# Autodesk Inventor assembly: STAGE1,ELEVATOR
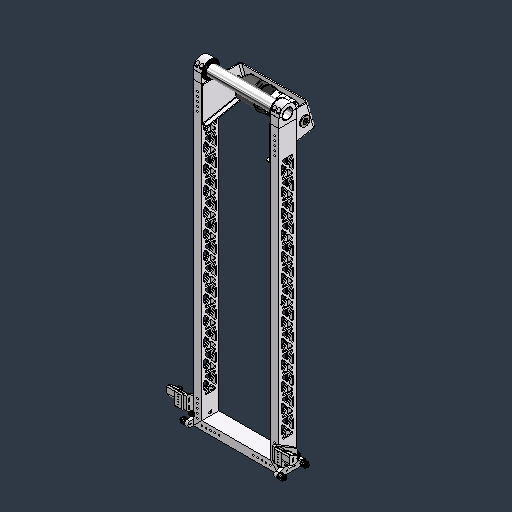
[picture p0: Inventor's stored thumbnail of the model, 512x512]
Saved by Autodesk Inventor 2024.3 (Build 283343000, 343)
## iProperties
ILogicPurgeVersion: 0.0.0.0
OnSaveVersion: 3.5.0.0
OnSaveAssembly: COREAutomationManager
Created: 2025-02-04
Part Number: STAGE1,ELEVATOR
Document SubType Name: Assembly
Designer: Jthib
Mfg Approved By: John.Thibert
Mass: 2890.66 g
Surface Area: 6308.95 cm^2
Volume: 985.653 cm^3
Density: 2.93273 g/cm^3
ModelCat: Uncategorized
CN_MASS: 2.89
Author: Jthib
## Documents named in this file (22)
- D:\Inventor Projects\Poseidon V2\STAGE1,ELEVATOR.iam
- D:\Inventor Projects\Poseidon V2\TUBE,ELEVATOR,SIDE,STAGE1.ipt
- D:\Inventor Projects\Poseidon V2\TUBE,ELEVATOR,BOT,STAGE1.ipt
- D:\Inventor Projects\Poseidon V2\PLATE,BRACKET,ELEVATOR,STAGE1.ipt
- D:\Inventor Projects\Poseidon V2\SLIDE,ELEVATOR,STAGE1,LH.iam
- D:\Inventor Projects\Poseidon V2\SLIDE,ELEVATOR,STAGE1,RH.iam
- D:\Inventor Projects\Poseidon V2\BRACE,CHAIN,#25,ELEVATOR.ipt
- D:\Inventor Projects\Poseidon V2\60355K336_Ball Bearing.ipt
- D:\Inventor Projects\Poseidon V2\91259A171_Alloy Steel Shoulder Screw.ipt
- D:\Inventor Projects\Poseidon V2\BEARING,MOUNT,SIDE,ELEVATOR,MIRR.ipt
- D:\Inventor Projects\Poseidon V2\BEARING,MOUNT,SIDE,ELEVATOR.ipt
- D:\Inventor Projects\Poseidon V2\BLOCK,BEARING,ARM,ELEVATOR.ipt
- D:\Inventor Projects\Poseidon V2\TOP,BEARING_BLOCK,ELEVATOR.ipt
- D:\Inventor Projects\Poseidon V2\TUBE,AXLE,ARM.ipt
- D:\Inventor Projects\Poseidon V2\PLATE,CROSSBRACE,MOTOR,ARM.ipt
- D:\Inventor Projects\Poseidon V2\Purchased\5909K52_0.032 Thick Washer for 1-1-4 Shaft Diameter Needle-Roller Thrust Bearing\5909K52_0.032 Thick Washer for 1-1-4 Shaft Diameter Needle-Rol.ipt
- D:\Inventor Projects\Poseidon V2\Purchased\5909K38_Needle-Roller Thrust Bearing\5909K38_Needle-Roller Thrust Bearing\5909K38_Needle-Roller Thrust Bearing.ipt
- D:\Inventor Projects\Poseidon V2\PURCHASED,HEX_BEARING.ipt
- D:\Inventor Projects\Poseidon V2\#Poseidon 2025\Design Accelerator\Spur Gear13.ipt
- D:\Inventor Projects\Poseidon V2\VersaPlanetary v2 Dual Stage 10_1 with RS 550 (1).iam
- D:\Inventor Projects\Poseidon V2\CONTROLS,MOTOR,NEO,V1.ipt
- D:\Inventor Projects\Poseidon V2\1_CAD Library\PURCHASED,GEARBOX,VERSA_PLANETARY,ADAPTER_CIM.ipt
## Components (35 placed, 23 different names)
1. 5909K38_Needle-Roller Thrust Bearing:1
2. 5909K38_Needle-Roller Thrust Bearing:2
3. 5909K52_0.032 Thick Washer for 1-1-4 Shaft Diameter Needle-Rol:1
4. 5909K52_0.032 Thick Washer for 1-1-4 Shaft Diameter Needle-Rol:2
5. 5909K52_0.032 Thick Washer for 1-1-4 Shaft Diameter Needle-Rol:3
6. 5909K52_0.032 Thick Washer for 1-1-4 Shaft Diameter Needle-Rol:4
7. 60355K336_Ball Bearing:1
8. 60355K336_Ball Bearing:2
9. 91259A171_Alloy Steel Shoulder Screw:1
10. 91259A171_Alloy Steel Shoulder Screw:2
11. BEARING,MOUNT,SIDE,ELEVATOR,MIRR:1
12. BEARING,MOUNT,SIDE,ELEVATOR:1
13. BLOCK,BEARING,ARM,ELEVATOR:1 — Mate:51, Mate:52, Mate:53, Mate:54, Mate:58, Mate:59
14. BLOCK,BEARING,ARM,ELEVATOR:3 — Mate:55, Mate:56, Mate:57, Mate:60, Mate:61
15. BRACE,CHAIN,#25,ELEVATOR.ipt:1
16. BRACE,CHAIN,#25,ELEVATOR:2 — Mate:16, Mate:17, Mate:18
17. CONTROLS,MOTOR,NEO,V1:1
18. PLATE,BRACKET,ELEVATOR,STAGE1.ipt:1
19. PLATE,BRACKET,ELEVATOR,STAGE1.ipt:2 — Mate:42, Mate:44
20. PLATE,BRACKET,ELEVATOR,STAGE1:4 — Mate:19, Mate:20, Mate:48, Mate:49, Mate:50
21. PLATE,BRACKET,ELEVATOR,STAGE1:5 — Mate:22, Mate:23, Mate:41, Mate:43, Mate:45, Mate:47
22. PLATE,CROSSBRACE,MOTOR,ARM:1
23. PURCHASED,GEARBOX,VERSA_PLANETARY,ADAPTER_CIM:1
24. PURCHASED,HEX_BEARING:1 — Mate:80
25. SLIDE,ELEVATOR,STAGE1,LH.iam:1 [sub-assembly] — Mate:15, Mate:16, Mate:17, Mate:18
26. SLIDE,ELEVATOR,STAGE1,RH.iam:1 [sub-assembly] — Mate:46
27. Spur Gear1:1 — Mate:80
28. TOP,BEARING_BLOCK,ELEVATOR:1 — Mate:58, Mate:59
29. TOP,BEARING_BLOCK,ELEVATOR:2 — Mate:60, Mate:61
30. TUBE,AXLE,ARM:1
31. TUBE,ELEVATOR,BOT,STAGE1.ipt:1 — Mate:14, Mate:19, Mate:20, Mate:22, Mate:23, Mate:41, Mate:42
32. TUBE,ELEVATOR,SIDE,STAGE1.ipt:1 — Mate:13, Mate:48, Mate:49, Mate:50, Mate:51, Mate:52, Mate:53, Mate:54
33. TUBE,ELEVATOR,SIDE,STAGE1.ipt:2 — Mate:43, Mate:44, Mate:45, Mate:46, Mate:47, Mate:55, Mate:56, Mate:57
34. TUBE,AXLE,ARM:2
35. VersaPlanetary v2 Dual Stage 10_1 with RS 550 (1):1 [sub-assembly]
## Relationships (82: Mate 67, Insert 8, Tangent 4, Flush 3)
- [Insert]: PLATE,BRACKET,ELEVATOR,STAGE1.ipt:1 ↔ TUBE,ELEVATOR,BOT,STAGE1.ipt:1
- [Insert]: PLATE,BRACKET,ELEVATOR,STAGE1.ipt:1 ↔ TUBE,ELEVATOR,BOT,STAGE1.ipt:1
- [Insert]: PLATE,BRACKET,ELEVATOR,STAGE1.ipt:2 ↔ TUBE,ELEVATOR,BOT,STAGE1.ipt:1
- [Insert]: PLATE,BRACKET,ELEVATOR,STAGE1.ipt:2 ↔ TUBE,ELEVATOR,BOT,STAGE1.ipt:1
- [Mate]: SLIDE,ELEVATOR,STAGE1,RH.iam:1 ↔ TUBE,ELEVATOR,SIDE,STAGE1.ipt:2
- [Mate]: SLIDE,ELEVATOR,STAGE1,RH.iam:1 ↔ TUBE,ELEVATOR,SIDE,STAGE1.ipt:2
- [Mate]: SLIDE,ELEVATOR,STAGE1,LH.iam:1 ↔ TUBE,ELEVATOR,SIDE,STAGE1.ipt:1
- [Mate]: SLIDE,ELEVATOR,STAGE1,LH.iam:1 ↔ TUBE,ELEVATOR,SIDE,STAGE1.ipt:1
- [Mate]: BRACE,CHAIN,#25,ELEVATOR.ipt:1 ↔ SLIDE,ELEVATOR,STAGE1,RH.iam:1
- [Mate]: BRACE,CHAIN,#25,ELEVATOR.ipt:1 ↔ SLIDE,ELEVATOR,STAGE1,RH.iam:1
- [Mate]: BRACE,CHAIN,#25,ELEVATOR.ipt:1 ↔ SLIDE,ELEVATOR,STAGE1,RH.iam:1
- Mate:13 (-127 mm): TUBE,ELEVATOR,SIDE,STAGE1.ipt:1
- Mate:14 (-457.2 mm): TUBE,ELEVATOR,BOT,STAGE1.ipt:1
- Mate:15: SLIDE,ELEVATOR,STAGE1,LH.iam:1
- Mate:16: BRACE,CHAIN,#25,ELEVATOR:2 ↔ SLIDE,ELEVATOR,STAGE1,LH.iam:1
- Mate:17: BRACE,CHAIN,#25,ELEVATOR:2 ↔ SLIDE,ELEVATOR,STAGE1,LH.iam:1
- Mate:18: BRACE,CHAIN,#25,ELEVATOR:2 ↔ SLIDE,ELEVATOR,STAGE1,LH.iam:1
- Mate:19: PLATE,BRACKET,ELEVATOR,STAGE1:4 ↔ TUBE,ELEVATOR,BOT,STAGE1.ipt:1
- Mate:20: PLATE,BRACKET,ELEVATOR,STAGE1:4 ↔ TUBE,ELEVATOR,BOT,STAGE1.ipt:1
- Mate:22: PLATE,BRACKET,ELEVATOR,STAGE1:5 ↔ TUBE,ELEVATOR,BOT,STAGE1.ipt:1
- Mate:23: PLATE,BRACKET,ELEVATOR,STAGE1:5 ↔ TUBE,ELEVATOR,BOT,STAGE1.ipt:1
- [Mate]: 60355K336_Ball Bearing:1 ↔ 91259A171_Alloy Steel Shoulder Screw:1
- [Mate]: BEARING,MOUNT,SIDE,ELEVATOR,MIRR:1 ↔ BRACE,CHAIN,#25,ELEVATOR.ipt:1
- [Mate]: BEARING,MOUNT,SIDE,ELEVATOR,MIRR:1 ↔ BRACE,CHAIN,#25,ELEVATOR.ipt:1
- [Mate]: BEARING,MOUNT,SIDE,ELEVATOR,MIRR:1 ↔ BRACE,CHAIN,#25,ELEVATOR.ipt:1
- [Insert]: 60355K336_Ball Bearing:1 ↔ BEARING,MOUNT,SIDE,ELEVATOR,MIRR:1
- [Mate]: 60355K336_Ball Bearing:1 ↔ 91259A171_Alloy Steel Shoulder Screw:1
- [Mate]: 60355K336_Ball Bearing:2 ↔ 91259A171_Alloy Steel Shoulder Screw:2
- [Mate]: 60355K336_Ball Bearing:2 ↔ 91259A171_Alloy Steel Shoulder Screw:2
- [Insert]: 91259A171_Alloy Steel Shoulder Screw:2 ↔ BEARING,MOUNT,SIDE,ELEVATOR:1
- [Mate]: BEARING,MOUNT,SIDE,ELEVATOR:1 ↔ BRACE,CHAIN,#25,ELEVATOR:2
- [Mate]: BEARING,MOUNT,SIDE,ELEVATOR:1 ↔ BRACE,CHAIN,#25,ELEVATOR:2
- [Mate]: BEARING,MOUNT,SIDE,ELEVATOR:1 ↔ BRACE,CHAIN,#25,ELEVATOR:2
- Mate:41: PLATE,BRACKET,ELEVATOR,STAGE1:5 ↔ TUBE,ELEVATOR,BOT,STAGE1.ipt:1
- Mate:42: PLATE,BRACKET,ELEVATOR,STAGE1.ipt:2 ↔ TUBE,ELEVATOR,BOT,STAGE1.ipt:1
- Mate:43: PLATE,BRACKET,ELEVATOR,STAGE1:5 ↔ TUBE,ELEVATOR,SIDE,STAGE1.ipt:2
- Mate:44: PLATE,BRACKET,ELEVATOR,STAGE1.ipt:2 ↔ TUBE,ELEVATOR,SIDE,STAGE1.ipt:2
- Mate:45: PLATE,BRACKET,ELEVATOR,STAGE1:5 ↔ TUBE,ELEVATOR,SIDE,STAGE1.ipt:2
- Mate:46: SLIDE,ELEVATOR,STAGE1,RH.iam:1 ↔ TUBE,ELEVATOR,SIDE,STAGE1.ipt:2
- Mate:47: PLATE,BRACKET,ELEVATOR,STAGE1:5 ↔ TUBE,ELEVATOR,SIDE,STAGE1.ipt:2
- Mate:48: PLATE,BRACKET,ELEVATOR,STAGE1:4 ↔ TUBE,ELEVATOR,SIDE,STAGE1.ipt:1
- Mate:49: PLATE,BRACKET,ELEVATOR,STAGE1:4 ↔ TUBE,ELEVATOR,SIDE,STAGE1.ipt:1
- Mate:50: PLATE,BRACKET,ELEVATOR,STAGE1:4 ↔ TUBE,ELEVATOR,SIDE,STAGE1.ipt:1
- Mate:51: BLOCK,BEARING,ARM,ELEVATOR:1 ↔ TUBE,ELEVATOR,SIDE,STAGE1.ipt:1
- Mate:52: BLOCK,BEARING,ARM,ELEVATOR:1 ↔ TUBE,ELEVATOR,SIDE,STAGE1.ipt:1
- Mate:53: BLOCK,BEARING,ARM,ELEVATOR:1 ↔ TUBE,ELEVATOR,SIDE,STAGE1.ipt:1
- Mate:54: BLOCK,BEARING,ARM,ELEVATOR:1 ↔ TUBE,ELEVATOR,SIDE,STAGE1.ipt:1
- Mate:55: BLOCK,BEARING,ARM,ELEVATOR:3 ↔ TUBE,ELEVATOR,SIDE,STAGE1.ipt:2
- Mate:56: BLOCK,BEARING,ARM,ELEVATOR:3 ↔ TUBE,ELEVATOR,SIDE,STAGE1.ipt:2
- Mate:57: BLOCK,BEARING,ARM,ELEVATOR:3 ↔ TUBE,ELEVATOR,SIDE,STAGE1.ipt:2
- Mate:58: BLOCK,BEARING,ARM,ELEVATOR:1 ↔ TOP,BEARING_BLOCK,ELEVATOR:1
- Mate:59: BLOCK,BEARING,ARM,ELEVATOR:1 ↔ TOP,BEARING_BLOCK,ELEVATOR:1
- Mate:60: BLOCK,BEARING,ARM,ELEVATOR:3 ↔ TOP,BEARING_BLOCK,ELEVATOR:2
- Mate:61: BLOCK,BEARING,ARM,ELEVATOR:3 ↔ TOP,BEARING_BLOCK,ELEVATOR:2
- [Mate]: BLOCK,BEARING,ARM,ELEVATOR:3 ↔ TUBE,AXLE,ARM:1
- [Flush]: TOP,BEARING_BLOCK,ELEVATOR:1 ↔ TUBE,AXLE,ARM:1
- [Mate]: PLATE,CROSSBRACE,MOTOR,ARM:1 ↔ TUBE,ELEVATOR,SIDE,STAGE1.ipt:1
- [Mate]: PLATE,CROSSBRACE,MOTOR,ARM:1 ↔ TUBE,ELEVATOR,SIDE,STAGE1.ipt:1
- [Flush]: PLATE,CROSSBRACE,MOTOR,ARM:1 ↔ TUBE,ELEVATOR,SIDE,STAGE1.ipt:1
- [Tangent]: 5909K38_Needle-Roller Thrust Bearing:1 ↔ 5909K52_0.032 Thick Washer for 1-1-4 Shaft Diameter Needle-Rol:1
- [Tangent]: 5909K38_Needle-Roller Thrust Bearing:1 ↔ 5909K52_0.032 Thick Washer for 1-1-4 Shaft Diameter Needle-Rol:2
- [Tangent]: 5909K38_Needle-Roller Thrust Bearing:2 ↔ 5909K52_0.032 Thick Washer for 1-1-4 Shaft Diameter Needle-Rol:3
- [Tangent]: 5909K38_Needle-Roller Thrust Bearing:2 ↔ 5909K52_0.032 Thick Washer for 1-1-4 Shaft Diameter Needle-Rol:4
- [Mate]: 5909K52_0.032 Thick Washer for 1-1-4 Shaft Diameter Needle-Rol:3 ↔ TOP,BEARING_BLOCK,ELEVATOR:2
- [Insert]: PLATE,CROSSBRACE,MOTOR,ARM:1 ↔ PURCHASED,HEX_BEARING:1
- [Insert]: CONTROLS,MOTOR,NEO,V1:1 ↔ PURCHASED,GEARBOX,VERSA_PLANETARY,ADAPTER_CIM:1
- [Mate]: CONTROLS,MOTOR,NEO,V1:1 ↔ VersaPlanetary v2 Dual Stage 10_1 with RS 550 (1):1
- [Mate]: PLATE,CROSSBRACE,MOTOR,ARM:1 ↔ VersaPlanetary v2 Dual Stage 10_1 with RS 550 (1):1
- [Mate]: PURCHASED,GEARBOX,VERSA_PLANETARY,ADAPTER_CIM:1 ↔ VersaPlanetary v2 Dual Stage 10_1 with RS 550 (1):1
- [Mate]: PLATE,CROSSBRACE,MOTOR,ARM:1 ↔ VersaPlanetary v2 Dual Stage 10_1 with RS 550 (1):1
- [Mate]: CONTROLS,MOTOR,NEO,V1:1 ↔ PURCHASED,GEARBOX,VERSA_PLANETARY,ADAPTER_CIM:1
- [Mate]: Spur Gear1:1 ↔ VersaPlanetary v2 Dual Stage 10_1 with RS 550 (1):1
- [Mate]: PLATE,CROSSBRACE,MOTOR,ARM:1 ↔ VersaPlanetary v2 Dual Stage 10_1 with RS 550 (1):1
- [Mate]: BLOCK,BEARING,ARM,ELEVATOR:3 ↔ TUBE,AXLE,ARM:2
- [Flush]: TOP,BEARING_BLOCK,ELEVATOR:1 ↔ TUBE,AXLE,ARM:2
- [Mate]: 5909K52_0.032 Thick Washer for 1-1-4 Shaft Diameter Needle-Rol:1 ↔ TUBE,AXLE,ARM:2
- [Mate]: 5909K38_Needle-Roller Thrust Bearing:1 ↔ TUBE,AXLE,ARM:2
- [Mate]: 5909K52_0.032 Thick Washer for 1-1-4 Shaft Diameter Needle-Rol:2 ↔ TUBE,AXLE,ARM:2
- [Mate]: 5909K52_0.032 Thick Washer for 1-1-4 Shaft Diameter Needle-Rol:3 ↔ TUBE,AXLE,ARM:2
- [Mate]: 5909K38_Needle-Roller Thrust Bearing:2 ↔ TUBE,AXLE,ARM:2
- [Mate]: 5909K52_0.032 Thick Washer for 1-1-4 Shaft Diameter Needle-Rol:4 ↔ TUBE,AXLE,ARM:2
- Mate:80: PURCHASED,HEX_BEARING:1 ↔ Spur Gear1:1
## Named parameters: d1097_d52 = 0 mm, d1156_d1097_d52 = 0 mm, d1158_d1102 = 0 mm, d1291_d1288 = 0 mm, d1292_d1290 = 0 mm, d1183_d1175 = 0 mm, d1185_d1182 = 0 mm, d140_d1164 = 0 mm, d141_d1165 = 0 mm
